# Autodesk Inventor assembly: climber
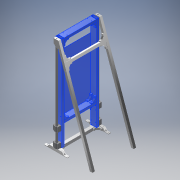
[picture p0: Inventor's stored thumbnail of the model, 180x180]
Saved by Autodesk Inventor 2019.4 (Build 234330000, 330)
## iProperties
Created: 2020-01-07
Part Number: climber
Document SubType Name: Assembly
Designer: Mark
Mass: 11763.3 g
Surface Area: 18434.4 cm^2
Volume: 3352.28 cm^3
Density: 3.50905 g/cm^3
Author: Mark
## Documents named in this file (10)
- C:\Users\Mark\Desktop\7738 Helion Engineering\7738-2020\Elevator Mechanism\climber.iam
- C:\Users\Mark\Desktop\7738 Helion Engineering\7738-2020\Elevator Mechanism\Extrusion Mid.ipt
- C:\Users\Mark\Desktop\7738 Helion Engineering\7738-2020\Elevator Mechanism\climber\Design Accelerator\Shaft2.iam
- C:\Users\Mark\Desktop\7738 Helion Engineering\7738-2020\Elevator Mechanism\Base.ipt
- C:\Users\Mark\Desktop\7738 Helion Engineering\7738-2020\Elevator Mechanism\Standard Bracing.ipt
- C:\Users\Mark\Desktop\7738 Helion Engineering\7738-2020\Elevator Mechanism\Top Connector.ipt
- C:\Users\Mark\Desktop\7738 Helion Engineering\7738-2020\Elevator Mechanism\Elevator Support.ipt
- C:\Users\Mark\Desktop\7738 Helion Engineering\7738-2020\Elevator Mechanism\Top Support.ipt
- C:\Users\Mark\Desktop\7738 Helion Engineering\7738-2020\Elevator Mechanism\Lifting Part.iam
- C:\Users\Mark\Desktop\7738 Helion Engineering\7738-2020\Elevator Mechanism\Линейный подшипник SCS 20UU.ipt
## Components (23 placed, 9 different names)
1. Extrusion Mid:1 — Mate:10, Flush:3, Flush:4, Mate:50, Mate:65, Mate:67, Mate:69, Mate:70, Mate:72, Mate:73
2. Shaft:1 [sub-assembly] — Mate:7, Mate:8, Mate:20, Mate:21, Mate:39, Mate:40
3. Shaft:2 [sub-assembly] — Mate:6, Flush:1, Mate:26, Mate:27, Cylindrical:1, Mate:52
4. Base:1 — Mate:6, Flush:1, Mate:9, Flush:2, Mate:10, Flush:3, Flush:4, Flush:5, Flush:16, Mate:64, Mate:66, Mate:68
5. Base:2 — Mate:7, Mate:8, Mate:9, Flush:2, Flush:5, Flush:6, Flush:7, Mate:51, Mate:71, Mate:74, Mate:75
6. Standard Bracing:1 — Mate:73, Mate:74, Mate:75
7. Standard Bracing:2 — Mate:70, Mate:71, Mate:72
8. Standard Bracing:3 — Mate:67, Mate:68, Mate:69
9. Standard Bracing:4 — Mate:64, Mate:65, Mate:66
10. Top Connector:1 — Mate:20, Flush:6, Mate:21, Flush:7, Flush:8, Mate:59, Mate:60
11. Elevator Support:1 — Flush:8, Mate:28, Flush:11, Mate:36, Mate:37, Mate:59, Mate:60
12. Top Connector:2 — Mate:26, Mate:27, Mate:57, Mate:58
13. Elevator Support:2 — Mate:57, Flush:16, Mate:58, Mate:62, Mate:63, Flush:17
14. Top Support:1 — Mate:28, Flush:11, Mate:31, Mate:32, Mate:33, Mate:38, Mate:61
15. Standard Bracing:5 — Mate:32, Mate:33, Mate:62
16. Standard Bracing:6 — Mate:31, Mate:63, Flush:17
17. Standard Bracing:7 — Flush:12, Mate:35, Flush:13
18. Standard Bracing:8 — Flush:12, Mate:35, Flush:13, Mate:36, Mate:37, Mate:38, Mate:61
19. Lifting Part:1 [sub-assembly] — Mate:53, Mate:54, Flush:15, Mate:55, Mate:56
20. Линейный подшипник SCS 20UU:1 — Mate:39, Mate:56
21. Линейный подшипник SCS 20UU:2 — Mate:40, Mate:55
22. Линейный подшипник SCS 20UU:3 — Mate:43, Flush:14, Cylindrical:1
23. Линейный подшипник SCS 20UU:4 — Mate:43, Flush:14, Mate:52, Mate:53, Mate:54, Flush:15
## Relationships (62: Mate 46, Flush 15, CylindricalJoint 1)
- Mate:6: Shaft:2 ↔ Base:1
- Flush:1: Shaft:2 ↔ Base:1
- Mate:7: Shaft:1 ↔ Base:2
- Mate:8: Shaft:1 ↔ Base:2
- Mate:9 (400 mm): Base:1 ↔ Base:2
- Flush:2: Base:1 ↔ Base:2
- Mate:10: Extrusion Mid:1 ↔ Base:1
- Flush:3: Extrusion Mid:1 ↔ Base:1
- Flush:4 (100 mm): Extrusion Mid:1 ↔ Base:1
- Flush:5: Base:1 ↔ Base:2
- Mate:20: Shaft:1 ↔ Top Connector:1
- Flush:6: Base:2 ↔ Top Connector:1
- Mate:21: Shaft:1 ↔ Top Connector:1
- Flush:7: Base:2 ↔ Top Connector:1
- Flush:8: Top Connector:1 ↔ Elevator Support:1
- Mate:26: Shaft:2 ↔ Top Connector:2
- Mate:27: Shaft:2 ↔ Top Connector:2
- Mate:28: Elevator Support:1 ↔ Top Support:1
- Flush:11: Elevator Support:1 ↔ Top Support:1
- Mate:31: Top Support:1 ↔ Standard Bracing:6
- Mate:32: Top Support:1 ↔ Standard Bracing:5
- Mate:33: Top Support:1 ↔ Standard Bracing:5
- Flush:12: Standard Bracing:7 ↔ Standard Bracing:8
- Mate:35 (25 mm): Standard Bracing:7 ↔ Standard Bracing:8
- Flush:13: Standard Bracing:7 ↔ Standard Bracing:8
- Mate:36: Elevator Support:1 ↔ Standard Bracing:8
- Mate:37: Elevator Support:1 ↔ Standard Bracing:8
- Mate:38: Top Support:1 ↔ Standard Bracing:8
- Mate:39: Shaft:1 ↔ Линейный подшипник SCS 20UU:1
- Mate:40: Shaft:1 ↔ Линейный подшипник SCS 20UU:2
- Mate:43 (100 mm): Линейный подшипник SCS 20UU:3 ↔ Линейный подшипник SCS 20UU:4
- Flush:14: Линейный подшипник SCS 20UU:3 ↔ Линейный подшипник SCS 20UU:4
- Cylindrical:1: Shaft:2 ↔ Линейный подшипник SCS 20UU:3
- Mate:50: Extrusion Mid:1
- Mate:51: Base:2
- Mate:52: Shaft:2 ↔ Линейный подшипник SCS 20UU:4
- Mate:53: Lifting Part:1 ↔ Линейный подшипник SCS 20UU:4
- Mate:54: Lifting Part:1 ↔ Линейный подшипник SCS 20UU:4
- Flush:15: Lifting Part:1 ↔ Линейный подшипник SCS 20UU:4
- Mate:55: Lifting Part:1 ↔ Линейный подшипник SCS 20UU:2
- Mate:56: Lifting Part:1 ↔ Линейный подшипник SCS 20UU:1
- Mate:57: Top Connector:2 ↔ Elevator Support:2
- Flush:16: Base:1 ↔ Elevator Support:2
- Mate:58: Top Connector:2 ↔ Elevator Support:2
- Mate:59: Top Connector:1 ↔ Elevator Support:1
- Mate:60: Top Connector:1 ↔ Elevator Support:1
- Mate:61: Top Support:1 ↔ Standard Bracing:8
- Mate:62: Elevator Support:2 ↔ Standard Bracing:5
- Mate:63: Elevator Support:2 ↔ Standard Bracing:6
- Flush:17: Elevator Support:2 ↔ Standard Bracing:6
- Mate:64: Base:1 ↔ Standard Bracing:4
- Mate:65: Extrusion Mid:1 ↔ Standard Bracing:4
- Mate:66: Base:1 ↔ Standard Bracing:4
- Mate:67: Extrusion Mid:1 ↔ Standard Bracing:3
- Mate:68: Base:1 ↔ Standard Bracing:3
- Mate:69: Extrusion Mid:1 ↔ Standard Bracing:3
- Mate:70: Extrusion Mid:1 ↔ Standard Bracing:2
- Mate:71: Base:2 ↔ Standard Bracing:2
- Mate:72: Extrusion Mid:1 ↔ Standard Bracing:2
- Mate:73: Extrusion Mid:1 ↔ Standard Bracing:1
- Mate:74: Base:2 ↔ Standard Bracing:1
- Mate:75: Base:2 ↔ Standard Bracing:1
